# Autodesk Inventor assembly: rack_and_pinion
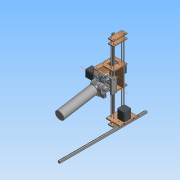
[picture p0: Inventor's stored thumbnail of the model, 180x180]
Saved by Autodesk Inventor 2015 (Build 190159000, 159)
## iProperties
Created: 2014-09-02
Part Number: rack_and_pinion
Document SubType Name: Assembly
Designer: shohei
Author: shohei
## Documents named in this file (14)
- C:\Users\shohei\Documents\Inventor\PlasmaCNCrev3\Workspaces\Workspace\rack_and_pinion.iam
- C:\Users\shohei\Documents\Inventor\PlasmaCNCrev3\Workspaces\Workspace\rack1.ipt
- C:\Users\shohei\Documents\Inventor\PlasmaCNCrev3\Workspaces\Workspace\rack_and_pinion\Design Accelerator\Spur Gears1.iam
- C:\Users\shohei\Documents\Inventor\PlasmaCNCrev3\Workspaces\Workspace\42BYGHM809.ipt
- C:\Users\shohei\Documents\Inventor\PlasmaCNCrev3\Workspaces\Workspace\holder_plate.ipt
- C:\Users\shohei\Documents\Inventor\PlasmaCNCrev3\Workspaces\Workspace\rack_and_pinion_X.iam
- C:\Users\shohei\Documents\Inventor\PlasmaCNCrev3\Workspaces\Workspace\longshaft.ipt
- C:\Users\shohei\Documents\Inventor\PlasmaCNCrev3\Workspaces\Workspace\torchHolder.ipt
- C:\Users\shohei\Documents\Inventor\PlasmaCNCrev3\Workspaces\Workspace\holdersupport.ipt
- C:\Users\shohei\Documents\Inventor\PlasmaCNCrev3\Workspaces\Workspace\main\motor_assembly_z.iam
- C:\Users\shohei\Documents\Inventor\PlasmaCNCrev3\Workspaces\Workspace\holder_sideblock.ipt
- C:\Users\shohei\Documents\Inventor\PlasmaCNCrev3\Workspaces\Workspace\plasmaTorchAssembly.iam
- C:\Users\shohei\Documents\Inventor\PlasmaCNCrev3\Workspaces\Workspace\stopper.ipt
- C:\Users\shohei\Documents\Inventor\PlasmaCNCrev3\Workspaces\Workspace\holder_plate4.ipt
## Components (26 placed, 13 different names)
1. rack1:1 — Angle:1, Mate:4, Angle:3, Rotation/Translation:1, Angle:6, Tangent:1, Flush:55
2. Spur Gears:1 [sub-assembly] — Mate:1, Mate:2, Rotation/Translation:1, Mate:5, Angle:4, Tangent:1, Rotational:1, Flush:55
3. 42BYGHM809:1 — Rotational:1, Mate:47, Mate:48, Mate:81
4. holder_plate:1 — Mate:47, Mate:48, Flush:69, Mate:72, Flush:75, Cylindrical:47, Mate:81, Cylindrical:52
5. rack_and_pinion_X:1 [sub-assembly] — Rotational:8, Flush:69, Mate:72, Flush:75
6. longshaft:1 — Flush:67, Flush:74, Cylindrical:36, Cylindrical:38, Cylindrical:49
7. longshaft:2 — Flush:67, Flush:68, Cylindrical:35, Cylindrical:37, Cylindrical:47, Cylindrical:48, Cylindrical:50
8. 42BYGHM809:2 — Rotational:8, Angle:12, Mate:12, Mate:13, Mate:14
9. torchHolder:1 — Rotational:14, Insert:1, Angle:14, Insert:2, Angle:15, Insert:3, Angle:16, Insert:4, Angle:17, Angle:18
10. torchHolder:2 — Mate:54, Flush:65, Flush:66
11. holder_plate:3 — Mate:12, Mate:13, Mate:14, Mate:40, Mate:66, Mate:82
12. holdersupport:1 — Mate:40, Mate:46, Flush:54, Cylindrical:50, Rigid:1
13. holdersupport:2 — Mate:67, Flush:70, Flush:78, Flush:79
14. motor_assembly_z:1 [sub-assembly] — Mate:46, Flush:54, Mate:55, Mate:56, Mate:57, Mate:58, Mate:60, Mate:61, Mate:62, Mate:63, Mate:66, Mate:67, Flush:70, Flush:78, Flush:79, Mate:82
15. longshaft:3 — Flush:68, Rigid:1
16. holder_sideblock:1 — Insert:1, Angle:14, Mate:59
17. holder_sideblock:2 — Insert:3, Angle:16, Mate:56, Mate:57
18. holder_sideblock:3 — Insert:4, Angle:17
19. holder_sideblock:4 — Mate:54, Flush:65, Flush:66, Insert:2, Angle:15, Mate:55
20. plasmaTorchAssembly:1 [sub-assembly] — Rotational:14
21. stopper:2 — Mate:58, Mate:59, Mate:60
22. stopper:3 — Mate:61, Mate:62, Mate:63
23. holder_plate4:1 — Cylindrical:36, Cylindrical:37
24. holder_plate4:3 — Cylindrical:35, Cylindrical:38
25. longshaft:4 — Flush:74, Cylindrical:51, Cylindrical:52
26. holder_plate4:5 — Cylindrical:48, Cylindrical:49, Cylindrical:51
## Relationships (70: Mate 27, Flush 12, Angle 11, CylindricalJoint 10, Insert 4, RevoluteJoint 3, RelateRotateTranslate 1, Tangent 1, WeldJoint 1)
- Mate:1: Spur Gears:1
- Mate:2: Spur Gears:1
- Angle:1 (180 deg): rack1:1
- Mate:4: rack1:1
- Angle:3 (0 deg): rack1:1
- Rotation/Translation:1 [RelateRotateTranslate] (47.1239 mm): rack1:1 ↔ Spur Gears:1
- Mate:5: Spur Gears:1
- Angle:4 (12 deg): Spur Gears:1
- Angle:6 (0 deg): rack1:1
- Angle:7 (0 deg)
- Mate:6
- Tangent:1: rack1:1 ↔ Spur Gears:1
- Rotational:1 [RevoluteJoint]: Spur Gears:1 ↔ 42BYGHM809:1
- Rotational:8 [RevoluteJoint]: rack_and_pinion_X:1 ↔ 42BYGHM809:2
- Angle:12 (0 deg): 42BYGHM809:2
- Mate:12: 42BYGHM809:2 ↔ holder_plate:3
- Mate:13: 42BYGHM809:2 ↔ holder_plate:3
- Mate:14: 42BYGHM809:2 ↔ holder_plate:3
- Mate:40: holder_plate:3 ↔ holdersupport:1
- Mate:46: holdersupport:1 ↔ motor_assembly_z:1
- Flush:54: holdersupport:1 ↔ motor_assembly_z:1
- Flush:55: rack1:1 ↔ Spur Gears:1
- Mate:47: 42BYGHM809:1 ↔ holder_plate:1
- Mate:48: 42BYGHM809:1 ↔ holder_plate:1
- Mate:54: torchHolder:2 ↔ holder_sideblock:4
- Flush:65: torchHolder:2 ↔ holder_sideblock:4
- Flush:66: torchHolder:2 ↔ holder_sideblock:4
- Rotational:14 [RevoluteJoint]: torchHolder:1 ↔ plasmaTorchAssembly:1
- Insert:1: torchHolder:1 ↔ holder_sideblock:1
- Angle:14 (0 deg): torchHolder:1 ↔ holder_sideblock:1
- Insert:2: torchHolder:1 ↔ holder_sideblock:4
- Angle:15 (0 deg): torchHolder:1 ↔ holder_sideblock:4
- Insert:3: torchHolder:1 ↔ holder_sideblock:2
- Angle:16 (0 deg): torchHolder:1 ↔ holder_sideblock:2
- Insert:4: torchHolder:1 ↔ holder_sideblock:3
- Angle:17 (0 deg): torchHolder:1 ↔ holder_sideblock:3
- Angle:18 (0 deg): torchHolder:1
- Mate:55: motor_assembly_z:1 ↔ holder_sideblock:4
- Mate:56: motor_assembly_z:1 ↔ holder_sideblock:2
- Mate:57: motor_assembly_z:1 ↔ holder_sideblock:2
- Mate:58: motor_assembly_z:1 ↔ stopper:2
- Mate:59: holder_sideblock:1 ↔ stopper:2
- Mate:60: motor_assembly_z:1 ↔ stopper:2
- Mate:61: motor_assembly_z:1 ↔ stopper:3
- Mate:62: motor_assembly_z:1 ↔ stopper:3
- Mate:63: motor_assembly_z:1 ↔ stopper:3
- Flush:67: longshaft:1 ↔ longshaft:2
- Flush:68: longshaft:2 ↔ longshaft:3
- Flush:69: holder_plate:1 ↔ rack_and_pinion_X:1
- Mate:66: holder_plate:3 ↔ motor_assembly_z:1
- Mate:67: holdersupport:2 ↔ motor_assembly_z:1
- Flush:70: holdersupport:2 ↔ motor_assembly_z:1
- Flush:74: longshaft:1 ↔ longshaft:4
- Cylindrical:35: longshaft:2 ↔ holder_plate4:3
- Cylindrical:36: longshaft:1 ↔ holder_plate4:1
- Cylindrical:37: longshaft:2 ↔ holder_plate4:1
- Cylindrical:38: longshaft:1 ↔ holder_plate4:3
- Mate:72: holder_plate:1 ↔ rack_and_pinion_X:1
- Flush:75: holder_plate:1 ↔ rack_and_pinion_X:1
- Flush:78: holdersupport:2 ↔ motor_assembly_z:1
- Flush:79: holdersupport:2 ↔ motor_assembly_z:1
- Cylindrical:47: holder_plate:1 ↔ longshaft:2
- Mate:81: 42BYGHM809:1 ↔ holder_plate:1
- Cylindrical:48: longshaft:2 ↔ holder_plate4:5
- Cylindrical:49: longshaft:1 ↔ holder_plate4:5
- Cylindrical:50: longshaft:2 ↔ holdersupport:1
- Rigid:1 [WeldJoint]: holdersupport:1 ↔ longshaft:3
- Cylindrical:51: longshaft:4 ↔ holder_plate4:5
- Cylindrical:52: holder_plate:1 ↔ longshaft:4
- Mate:82: holder_plate:3 ↔ motor_assembly_z:1
